# Autodesk Inventor assembly: сборка акб
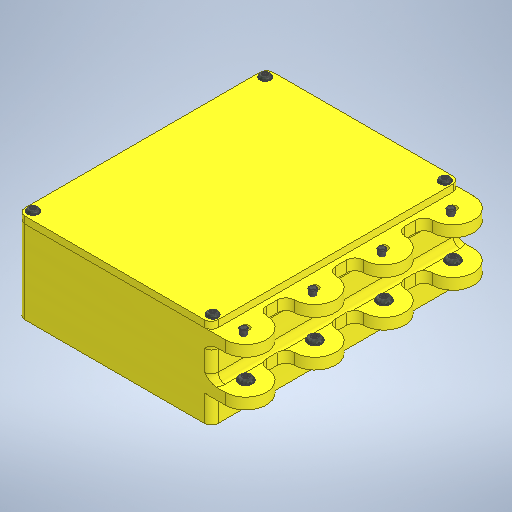
[picture p0: Inventor's stored thumbnail of the model, 512x512]
Saved by Autodesk Inventor 2025 (Build 290162000, 162)
## iProperties
Created: 2025-02-26
Part Number: сборка акб
Document SubType Name: Assembly
Designer: volko
Mass: 2307.29 g
Surface Area: 2403.39 cm^2
Volume: 1377.08 cm^3
Density: 1.6755 g/cm^3
Author: volko
## Documents named in this file (7)
- C:\Users\volko\Desktop\диплом\Модели\детали\сборка акб.iam
- C:\Users\volko\Desktop\диплом\Модели\детали\акб корпус.ipt
- C:\Users\volko\Desktop\диплом\Модели\детали\акб.ipt
- C:\Users\volko\Desktop\диплом\Модели\детали\акб_MIR.ipt
- C:\Users\volko\Desktop\диплом\Модели\детали\крышка акб.ipt
- C:\Users\volko\Desktop\диплом\Модели\детали\стандартные изделия\ru-RU\ISO 7380-1\ISO 7380-1 - M4 x 10.ipt
- C:\Users\volko\Desktop\диплом\Модели\детали\стандартные изделия\ru-RU\ISO 7380-1\ISO 7380-1 - M5 x 12.ipt
## Components (16 placed, 6 different names)
1. акб корпус:1 — Заподлицо:1, Заподлицо:2, Заподлицо:3, Совмещение:1, Заподлицо:4, Совмещение:2, Совмещение:3, Совмещение:6, Совмещение:7, Совмещение:9, Совмещение:10, Заподлицо:6, Совмещение:11
2. акб:1 — Совмещение:1, Заподлицо:4, Совмещение:2, Симметрия:1
3. акб_MIR:1 — Симметрия:1, Совмещение:3, Совмещение:4
4. крышка акб:1 — Совмещение:5, Совмещение:6, Заподлицо:5, Совмещение:8
5. ISO 7380-1 M4 x 10:2 — Совмещение:7, Совмещение:8
6. ISO 7380-1 M4 x 10:3
7. ISO 7380-1 M4 x 10:4
8. ISO 7380-1 M4 x 10:5
9. ISO 7380-1 M5 x 12:2 — Совмещение:11
10. ISO 7380-1 M5 x 12:1 — Совмещение:9, Совмещение:10
11. ISO 7380-1 M5 x 12:3
12. ISO 7380-1 M5 x 12:4
13. ISO 7380-1 M5 x 12:5
14. ISO 7380-1 M5 x 12:6
15. ISO 7380-1 M5 x 12:7
16. ISO 7380-1 M5 x 12:8
## Component patterns: (4 elements, first: ISO 7380-1 M4 x 10:2), (4 elements, first: ISO 7380-1 M5 x 12:2 + ISO 7380-1 M5 x 12:1)
## Relationships (18: Mate 11, Flush 6, Symmetry 1)
- Заподлицо:1 [Flush]: акб корпус:1
- Заподлицо:2 [Flush]: акб корпус:1
- Заподлицо:3 [Flush]: акб корпус:1
- Совмещение:1 [Mate]: акб корпус:1 ↔ акб:1
- Заподлицо:4 [Flush]: акб корпус:1 ↔ акб:1
- Совмещение:2 [Mate] (3.5 mm): акб корпус:1 ↔ акб:1
- Симметрия:1 [Symmetry]: акб:1 ↔ акб_MIR:1
- Совмещение:3 [Mate]: акб корпус:1 ↔ акб_MIR:1
- Совмещение:4 [Mate]: акб_MIR:1
- Совмещение:5 [Mate]: крышка акб:1
- Совмещение:6 [Mate]: акб корпус:1 ↔ крышка акб:1
- Заподлицо:5 [Flush]: крышка акб:1
- Совмещение:7 [Mate]: акб корпус:1 ↔ ISO 7380-1 M4 x 10:2
- Совмещение:8 [Mate]: крышка акб:1 ↔ ISO 7380-1 M4 x 10:2
- Совмещение:9 [Mate]: акб корпус:1 ↔ ISO 7380-1 M5 x 12:1
- Совмещение:10 [Mate]: акб корпус:1 ↔ ISO 7380-1 M5 x 12:1
- Заподлицо:6 [Flush] (12.5 mm): акб корпус:1
- Совмещение:11 [Mate]: акб корпус:1 ↔ ISO 7380-1 M5 x 12:2
